# Autodesk Inventor assembly: final billard car
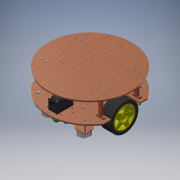
[picture p0: Inventor's stored thumbnail of the model, 180x180]
Saved by Autodesk Inventor 2017 (Build 210142000, 142)
## iProperties
Created: 2019-12-07
Part Number: final billard car
Document SubType Name: Assembly
Designer: User
Author: User
## Documents named in this file (21)
- D:\台大\大三上 108-1\機械設計\final billard car.iam
- D:\台大\大三上 108-1\機械設計\底盤.ipt
- D:\台大\大三上 108-1\機械設計\筷子套.ipt
- D:\台大\大三上 108-1\機械設計\筷子套軸.ipt
- D:\台大\大三上 108-1\機械設計\蓋子.ipt
- D:\台大\大三上 108-1\機械設計\蓋子2.ipt
- D:\台大\大三上 108-1\機械設計\轉軸.ipt
- D:\台大\大三上 108-1\機械設計\Servomotor.ipt
- D:\台大\大三上 108-1\機械設計\Servomotor-1.ipt
- D:\台大\大三上 108-1\機械設計\支架 assembly.ipt
- D:\台大\大三上 108-1\機械設計\DC motor.ipt
- D:\台大\大三上 108-1\機械設計\M2.ipt
- D:\台大\大三上 108-1\機械設計\輪胎.ipt
- D:\台大\大三上 108-1\機械設計\m3 nut.ipt
- D:\台大\大三上 108-1\機械設計\M3.ipt
- D:\台大\大三上 108-1\機械設計\M3-2.ipt
- D:\台大\大三上 108-1\機械設計\wheel2.ipt
- D:\台大\大三上 108-1\機械設計\shaft.ipt
- D:\台大\大三上 108-1\機械設計\second floor.ipt
- D:\台大\大三上 108-1\機械設計\sprimg.ipt
- D:\台大\大三上 108-1\機械設計\Part1.ipt
## Components (86 placed, 20 different names)
1. 底盤:1 — Mate:22, Mate:23, Mate:24, Mate:25, Mate:26, Mate:27, Mate:28, Mate:47, Flush:6, Mate:48, Mate:50, Flush:7, Mate:61, Mate:62, Mate:63, Mate:64, Mate:67, Mate:68, Mate:72, Mate:75, Mate:76, Mate:80, Mate:89, Mate:90, Mate:95, Mate:96, Mate:98, Mate:99, Mate:100, Mate:107, Mate:108, Mate:114, Mate:118, Mate:119, Mate:124, Mate:127, Mate:131, Mate:132, Mate:133, Mate:135, Mate:138, Mate:142, Mate:144, Mate:145, Mate:146, Mate:147, Mate:149, Mate:151, Mate:155, Mate:157, Mate:163, Mate:165, Mate:170, Mate:171, Mate:172, Mate:173, Mate:174, Mate:175, Mate:180, Mate:181, Mate:182, Mate:183
2. 蓋子:1 — Mate:6, Flush:2
3. 蓋子2:1 — Mate:6, Flush:2, Mate:22, Mate:50, Flush:7, Mate:54
4. 支架 assembly:1 — Mate:23, Mate:24, Mate:25, Mate:29, Mate:30, Mate:32, Mate:34, Mate:35
5. 支架 assembly:2 — Mate:26, Mate:27, Mate:28, Mate:36, Mate:38, Mate:40, Mate:41, Mate:42
6. DC motor:1 — Mate:29, Mate:31, Mate:33, Mate:45, Mate:46
7. DC motor:2 — Mate:36, Mate:37, Mate:39, Mate:43, Mate:44
8. M2:1 — Mate:30, Mate:31, Mate:32
9. M2:2 — Mate:33, Mate:34, Mate:35
10. M2:3 — Mate:37, Mate:38, Mate:42
11. M2:4 — Mate:39, Mate:40, Mate:41
12. 輪胎:1 — Mate:45, Mate:46
13. 輪胎:2 — Mate:43, Mate:44
14. Servomotor:1 — Mate:59, Mate:61, Mate:62, Mate:63, Mate:64, Mate:65, Mate:66, Mate:70, Mate:71, Mate:73, Mate:77, Mate:79, Mate:82
15. Servomotor-1:1 — Mate:65, Mate:66
16. 筷子套:1 — Mate:54, Mate:55, Mate:134, Mate:226, Mate:228, Mate:230
17. 筷子套軸:1 — Mate:55, Mate:57, Mate:58, Mate:134, Mate:229, Mate:232
18. 轉軸:1 — Mate:57, Mate:58, Mate:59, Mate:231
19. m3 nut:1 — Mate:73, Mate:74
20. M3:1 — Mate:71, Mate:72, Mate:74
21. m3 nut:2 — Mate:81, Mate:82
22. M3:2 — Mate:79, Mate:80, Mate:81
23. m3 nut:3 — Mate:77, Mate:78
24. M3:3 — Mate:75, Mate:76, Mate:78
25. m3 nut:4 — Mate:69, Mate:70
26. M3:4 — Mate:67, Mate:68, Mate:69
27. m3 nut:5 — Mate:114, Mate:115
28. M3-2:1 — Mate:92, Mate:93, Mate:97, Mate:133
29. wheel2:1 — Mate:87, Mate:88, Mate:92, Mate:93, Mate:95
30. m3 nut:6 — Mate:107, Mate:110
31. M3-2:2 — Mate:103, Mate:104, Mate:109, Mate:131
32. wheel2:2 — Mate:98, Mate:136, Mate:137, Mate:141, Mate:143
33. m3 nut:7 — Mate:127, Mate:139
34. M3-2:3 — Mate:101, Mate:102, Mate:110, Mate:132
35. wheel2:3 — Mate:100, Mate:101, Mate:102, Mate:103, Mate:104
36. m3 nut:8 — Mate:108, Mate:109
37. M3-2:4 — Mate:111, Mate:112, Mate:115, Mate:135
38. wheel2:4 — Mate:99, Mate:111, Mate:112, Mate:116, Mate:117
39. m3 nut:9 — Mate:89, Mate:90, Mate:91
40. M3-2:5 — Mate:87, Mate:88, Mate:91
41. m3 nut:10 — Mate:119, Mate:120
42. M3-2:6 — Mate:140, Mate:141, Mate:142, Mate:143
43. m3 nut:11 — Mate:96, Mate:97
44. M3-2:7 — Mate:136, Mate:137, Mate:138, Mate:139
45. m3 nut:12 — Mate:124, Mate:140
46. M3-2:8 — Mate:116, Mate:117, Mate:118, Mate:120
47. shaft:1 — Mate:145, Mate:154, Mate:156, Mate:158, Mate:159, Mate:190, Mate:194, Mate:195, Mate:198
48. shaft:2 — Mate:146, Mate:160, Mate:161, Mate:162, Mate:164, Mate:188, Mate:206, Mate:224, Mate:225
49. shaft:3 — Mate:147, Mate:166, Mate:167, Mate:168, Mate:169, Mate:187, Mate:222, Mate:223
50. shaft:4 — Mate:144, Mate:148, Mate:150, Mate:152, Mate:153, Mate:199, Mate:201, Mate:202, Mate:220, Mate:221
51. m3 nut:13 — Mate:181, Mate:185
52. M3:5 — Mate:154, Mate:155, Mate:156, Mate:184
53. m3 nut:14 — Mate:183, Mate:186
54. M3:6 — Mate:157, Mate:158, Mate:159, Mate:185
55. m3 nut:15 — Mate:180, Mate:184
56. M3:7 — Mate:151, Mate:152, Mate:153, Mate:179
57. m3 nut:16 — Mate:182, Mate:187
58. M3:8 — Mate:160, Mate:162, Mate:163, Mate:176
59. m3 nut:17 — Mate:173, Mate:177
60. M3:9 — Mate:161, Mate:164, Mate:165, Mate:177
61. m3 nut:18 — Mate:172, Mate:176
62. M3:10 — Mate:148, Mate:149, Mate:150, Mate:178
63. m3 nut:19 — Mate:174, Mate:179
64. M3:11 — Mate:166, Mate:169, Mate:171
65. m3 nut:20 — Mate:175, Mate:178
66. M3:12 — Mate:167, Mate:168, Mate:170, Mate:186
67. second floor:1 — Mate:188, Mate:189, Mate:191, Mate:192, Mate:193, Mate:200, Mate:203, Mate:204, Mate:205, Mate:207, Mate:208, Mate:209, Mate:210, Mate:211, Mate:212, Mate:213
68. m3 nut:21 — Mate:195, Mate:196
69. M3:13 — Mate:199, Mate:200, Mate:201, Mate:219
70. m3 nut:22 — Mate:215, Mate:223
71. M3:14 — Mate:192, Mate:193, Mate:194, Mate:197
72. m3 nut:23 — Mate:197, Mate:198
73. M3:15 — Mate:189, Mate:190, Mate:191, Mate:196
74. m3 nut:24 — Mate:218, Mate:221
75. M3:16 — Mate:210, Mate:213, Mate:215
76. m3 nut:25 — Mate:214, Mate:222
77. M3:17 — Mate:205, Mate:206, Mate:207, Mate:217
78. m3 nut:26 — Mate:217, Mate:225
79. M3:18 — Mate:208, Mate:209, Mate:216
80. m3 nut:27 — Mate:216, Mate:224
81. M3:19 — Mate:202, Mate:203, Mate:204, Mate:218
82. m3 nut:28 — Mate:219, Mate:220
83. M3:20 — Mate:211, Mate:212, Mate:214
84. sprimg:1 — Mate:226, Mate:228
85. Part1:1 — Mate:231, Mate:232
86. Part1:2 — Mate:229, Mate:230
## Relationships (192: Mate 189, Flush 3)
- Mate:6: 蓋子:1 ↔ 蓋子2:1
- Flush:2: 蓋子:1 ↔ 蓋子2:1
- Mate:22: 底盤:1 ↔ 蓋子2:1
- Mate:23: 底盤:1 ↔ 支架 assembly:1
- Mate:24: 底盤:1 ↔ 支架 assembly:1
- Mate:25: 底盤:1 ↔ 支架 assembly:1
- Mate:26: 底盤:1 ↔ 支架 assembly:2
- Mate:27: 底盤:1 ↔ 支架 assembly:2
- Mate:28: 底盤:1 ↔ 支架 assembly:2
- Mate:29: 支架 assembly:1 ↔ DC motor:1
- Mate:30: 支架 assembly:1 ↔ M2:1
- Mate:31: DC motor:1 ↔ M2:1
- Mate:32: 支架 assembly:1 ↔ M2:1
- Mate:33: DC motor:1 ↔ M2:2
- Mate:34: 支架 assembly:1 ↔ M2:2
- Mate:35: 支架 assembly:1 ↔ M2:2
- Mate:36: 支架 assembly:2 ↔ DC motor:2
- Mate:37: DC motor:2 ↔ M2:3
- Mate:38: 支架 assembly:2 ↔ M2:3
- Mate:39: DC motor:2 ↔ M2:4
- Mate:40: 支架 assembly:2 ↔ M2:4
- Mate:41: 支架 assembly:2 ↔ M2:4
- Mate:42: 支架 assembly:2 ↔ M2:3
- Mate:43: DC motor:2 ↔ 輪胎:2
- Mate:44: DC motor:2 ↔ 輪胎:2
- Mate:45: DC motor:1 ↔ 輪胎:1
- Mate:46: DC motor:1 ↔ 輪胎:1
- Mate:47: 底盤:1
- Flush:6: 底盤:1
- Mate:48: 底盤:1
- Mate:50: 底盤:1 ↔ 蓋子2:1
- Flush:7 (-9 mm): 底盤:1 ↔ 蓋子2:1
- Mate:54: 蓋子2:1 ↔ 筷子套:1
- Mate:55: 筷子套:1 ↔ 筷子套軸:1
- Mate:57: 筷子套軸:1 ↔ 轉軸:1
- Mate:58: 筷子套軸:1 ↔ 轉軸:1
- Mate:59: Servomotor:1 ↔ 轉軸:1
- Mate:61: 底盤:1 ↔ Servomotor:1
- Mate:62: 底盤:1 ↔ Servomotor:1
- Mate:63: 底盤:1 ↔ Servomotor:1
- Mate:64: 底盤:1 ↔ Servomotor:1
- Mate:65: Servomotor:1 ↔ Servomotor-1:1
- Mate:66 (2 mm): Servomotor:1 ↔ Servomotor-1:1
- Mate:67: 底盤:1 ↔ M3:4
- Mate:68: 底盤:1 ↔ M3:4
- Mate:69: m3 nut:4 ↔ M3:4
- Mate:70: Servomotor:1 ↔ m3 nut:4
- Mate:71: Servomotor:1 ↔ M3:1
- Mate:72: 底盤:1 ↔ M3:1
- Mate:73: Servomotor:1 ↔ m3 nut:1
- Mate:74: m3 nut:1 ↔ M3:1
- Mate:75: 底盤:1 ↔ M3:3
- Mate:76: 底盤:1 ↔ M3:3
- Mate:77: Servomotor:1 ↔ m3 nut:3
- Mate:78: m3 nut:3 ↔ M3:3
- Mate:79: Servomotor:1 ↔ M3:2
- Mate:80: 底盤:1 ↔ M3:2
- Mate:81: m3 nut:2 ↔ M3:2
- Mate:82: Servomotor:1 ↔ m3 nut:2
- Mate:87: wheel2:1 ↔ M3-2:5
- Mate:88: wheel2:1 ↔ M3-2:5
- Mate:89: 底盤:1 ↔ m3 nut:9
- Mate:90: 底盤:1 ↔ m3 nut:9
- Mate:91: m3 nut:9 ↔ M3-2:5
- Mate:92: M3-2:1 ↔ wheel2:1
- Mate:93: M3-2:1 ↔ wheel2:1
- Mate:95 (21.25 mm): 底盤:1 ↔ wheel2:1
- Mate:96: 底盤:1 ↔ m3 nut:11
- Mate:97: M3-2:1 ↔ m3 nut:11
- Mate:98 (21.25 mm): 底盤:1 ↔ wheel2:2
- Mate:99 (21.25 mm): 底盤:1 ↔ wheel2:4
- Mate:100 (21.25 mm): 底盤:1 ↔ wheel2:3
- Mate:101: M3-2:3 ↔ wheel2:3
- Mate:102: M3-2:3 ↔ wheel2:3
- Mate:103: M3-2:2 ↔ wheel2:3
- Mate:104: M3-2:2 ↔ wheel2:3
- Mate:107: 底盤:1 ↔ m3 nut:6
- Mate:108: 底盤:1 ↔ m3 nut:8
- Mate:109: M3-2:2 ↔ m3 nut:8
- Mate:110: m3 nut:6 ↔ M3-2:3
- Mate:111: M3-2:4 ↔ wheel2:4
- Mate:112: M3-2:4 ↔ wheel2:4
- Mate:114: 底盤:1 ↔ m3 nut:5
- Mate:115: m3 nut:5 ↔ M3-2:4
- Mate:116: wheel2:4 ↔ M3-2:8
- Mate:117: wheel2:4 ↔ M3-2:8
- Mate:118: 底盤:1 ↔ M3-2:8
- Mate:119: 底盤:1 ↔ m3 nut:10
- Mate:120: m3 nut:10 ↔ M3-2:8
- Mate:124: 底盤:1 ↔ m3 nut:12
- Mate:127: 底盤:1 ↔ m3 nut:7
- Mate:131: 底盤:1 ↔ M3-2:2
- Mate:132: 底盤:1 ↔ M3-2:3
- Mate:133: 底盤:1 ↔ M3-2:1
- Mate:134: 筷子套:1 ↔ 筷子套軸:1
- Mate:135: 底盤:1 ↔ M3-2:4
- Mate:136: wheel2:2 ↔ M3-2:7
- Mate:137: wheel2:2 ↔ M3-2:7
- Mate:138: 底盤:1 ↔ M3-2:7
- Mate:139: m3 nut:7 ↔ M3-2:7
- Mate:140: M3-2:6 ↔ m3 nut:12
- Mate:141: wheel2:2 ↔ M3-2:6
- Mate:142: 底盤:1 ↔ M3-2:6
- Mate:143: wheel2:2 ↔ M3-2:6
- Mate:144: 底盤:1 ↔ shaft:4
- Mate:145: 底盤:1 ↔ shaft:1
- Mate:146: 底盤:1 ↔ shaft:2
- Mate:147: 底盤:1 ↔ shaft:3
- Mate:148: shaft:4 ↔ M3:10
- Mate:149: 底盤:1 ↔ M3:10
- Mate:150: shaft:4 ↔ M3:10
- Mate:151: 底盤:1 ↔ M3:7
- Mate:152: shaft:4 ↔ M3:7
- Mate:153: shaft:4 ↔ M3:7
- Mate:154: shaft:1 ↔ M3:5
- Mate:155: 底盤:1 ↔ M3:5
- Mate:156: shaft:1 ↔ M3:5
- Mate:157: 底盤:1 ↔ M3:6
- Mate:158: shaft:1 ↔ M3:6
- Mate:159: shaft:1 ↔ M3:6
- Mate:160: shaft:2 ↔ M3:8
- Mate:161: shaft:2 ↔ M3:9
- Mate:162: shaft:2 ↔ M3:8
- Mate:163: 底盤:1 ↔ M3:8
- Mate:164: shaft:2 ↔ M3:9
- Mate:165: 底盤:1 ↔ M3:9
- Mate:166: shaft:3 ↔ M3:11
- Mate:167: shaft:3 ↔ M3:12
- Mate:168: shaft:3 ↔ M3:12
- Mate:169: shaft:3 ↔ M3:11
- Mate:170: 底盤:1 ↔ M3:12
- Mate:171: 底盤:1 ↔ M3:11
- Mate:172: 底盤:1 ↔ m3 nut:18
- Mate:173: 底盤:1 ↔ m3 nut:17
- Mate:174: 底盤:1 ↔ m3 nut:19
- Mate:175: 底盤:1 ↔ m3 nut:20
- Mate:176: M3:8 ↔ m3 nut:18
- Mate:177: m3 nut:17 ↔ M3:9
- Mate:178: M3:10 ↔ m3 nut:20
- Mate:179: M3:7 ↔ m3 nut:19
- Mate:180: 底盤:1 ↔ m3 nut:15
- Mate:181: 底盤:1 ↔ m3 nut:13
- Mate:182: 底盤:1 ↔ m3 nut:16
- Mate:183: 底盤:1 ↔ m3 nut:14
- Mate:184: M3:5 ↔ m3 nut:15
- Mate:185: m3 nut:13 ↔ M3:6
- Mate:186: m3 nut:14 ↔ M3:12
- Mate:187: shaft:3 ↔ m3 nut:16
- Mate:188: shaft:2 ↔ second floor:1
- Mate:189: second floor:1 ↔ M3:15
- Mate:190: shaft:1 ↔ M3:15
- Mate:191: second floor:1 ↔ M3:15
- Mate:192: second floor:1 ↔ M3:14
- Mate:193: second floor:1 ↔ M3:14
- Mate:194: shaft:1 ↔ M3:14
- Mate:195: shaft:1 ↔ m3 nut:21
- Mate:196: m3 nut:21 ↔ M3:15
- Mate:197: M3:14 ↔ m3 nut:23
- Mate:198: shaft:1 ↔ m3 nut:23
- Mate:199: shaft:4 ↔ M3:13
- Mate:200: second floor:1 ↔ M3:13
- Mate:201: shaft:4 ↔ M3:13
- Mate:202: shaft:4 ↔ M3:19
- Mate:203: second floor:1 ↔ M3:19
- Mate:204: second floor:1 ↔ M3:19
- Mate:205: second floor:1 ↔ M3:17
- Mate:206: shaft:2 ↔ M3:17
- Mate:207: second floor:1 ↔ M3:17
- Mate:208: second floor:1 ↔ M3:18
- Mate:209: second floor:1 ↔ M3:18
- Mate:210: second floor:1 ↔ M3:16
- Mate:211: second floor:1 ↔ M3:20
- Mate:212: second floor:1 ↔ M3:20
- Mate:213: second floor:1 ↔ M3:16
- Mate:214: m3 nut:25 ↔ M3:20
- Mate:215: m3 nut:22 ↔ M3:16
- Mate:216: M3:18 ↔ m3 nut:27
- Mate:217: M3:17 ↔ m3 nut:26
- Mate:218: m3 nut:24 ↔ M3:19
- Mate:219: M3:13 ↔ m3 nut:28
- Mate:220: shaft:4 ↔ m3 nut:28
- Mate:221: shaft:4 ↔ m3 nut:24
- Mate:222: shaft:3 ↔ m3 nut:25
- Mate:223: shaft:3 ↔ m3 nut:22
- Mate:224: shaft:2 ↔ m3 nut:27
- Mate:225: shaft:2 ↔ m3 nut:26
- Mate:226: 筷子套:1 ↔ sprimg:1
- Mate:228: 筷子套:1 ↔ sprimg:1
- Mate:229: 筷子套軸:1 ↔ Part1:2
- Mate:230: 筷子套:1 ↔ Part1:2
- Mate:231: 轉軸:1 ↔ Part1:1
- Mate:232: 筷子套軸:1 ↔ Part1:1
